# Autodesk Inventor assembly: Body Cover Assembly
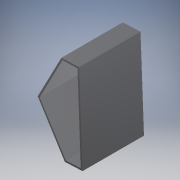
[picture p0: Inventor's stored thumbnail of the model, 180x180]
Saved by Autodesk Inventor 2017 (Build 210142000, 142)
## iProperties
Created: 2018-10-18
Part Number: Body Cover Assembly
Document SubType Name: Assembly
Designer: Dell
Author: Dell
## Documents named in this file (5)
- C:\Users\Dell\Documents\GitHub\tr2\Body\Body Cover Assembly.iam
- C:\Users\Dell\Documents\GitHub\tr2\Body\BO07.ipt
- C:\Users\Dell\Documents\GitHub\tr2\Body\BO08.ipt
- C:\Users\Dell\Documents\GitHub\tr2\Body\BO10.ipt
- C:\Users\Dell\Documents\GitHub\tr2\Body\BO11.ipt
## Components (6 placed, 4 different names)
1. BO07:1 — Flush:4, Mate:20, Mate:32, Mate:39
2. BO08:2 — Mate:29, Mate:32, Mate:33, Mate:38
3. BO08:3 — Mate:19, Flush:5
4. BO07:2 — Mate:19, Flush:4, Mate:20, Flush:5, Mate:36
5. BO10:1 — Mate:29, Mate:33, Flush:8, Mate:37
6. BO11:2 — Mate:36, Flush:8, Mate:37, Mate:38, Mate:39
## Relationships (12: Mate 9, Flush 3)
- Mate:19: BO08:3 ↔ BO07:2
- Flush:4: BO07:1 ↔ BO07:2
- Mate:20: BO07:1 ↔ BO07:2
- Flush:5: BO08:3 ↔ BO07:2
- Mate:29: BO08:2 ↔ BO10:1
- Mate:32: BO07:1 ↔ BO08:2
- Mate:33: BO08:2 ↔ BO10:1
- Mate:36: BO07:2 ↔ BO11:2
- Flush:8: BO10:1 ↔ BO11:2
- Mate:37: BO10:1 ↔ BO11:2
- Mate:38: BO08:2 ↔ BO11:2
- Mate:39: BO07:1 ↔ BO11:2
